# Autodesk Inventor assembly: Chassis Frame Layout
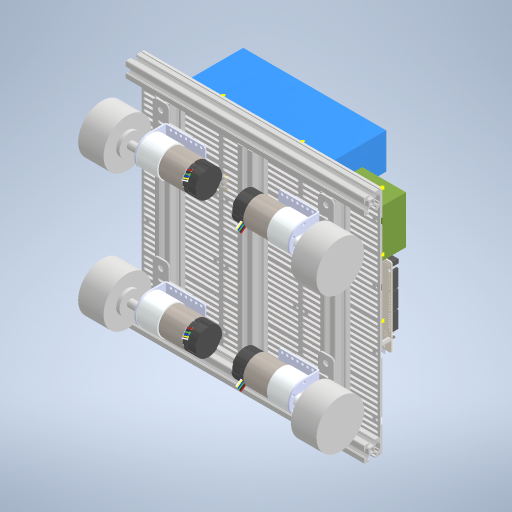
[picture p0: Inventor's stored thumbnail of the model, 512x512]
Saved by Autodesk Inventor 2024 (Build 280153000, 153)
## iProperties
Created: 2023-10-20
Part Number: Chassis Frame Layout
Document SubType Name: Assembly
Designer: olson
Author: olson
## Documents named in this file (20)
- C:\Users\olson\OneDrive\Documents\Senior Year\FALL 2023\ECE 4961 - Capstone 1\Detail Design\Chassis Frame\CAD Models\Chassis Frame Layout.iam
- C:\Users\olson\OneDrive\Documents\Senior Year\FALL 2023\ECE 4961 - Capstone 1\Detail Design\Chassis Frame\CAD Models\Extruded Alumnium 250mm.ipt
- C:\Users\olson\OneDrive\Documents\Senior Year\FALL 2023\ECE 4961 - Capstone 1\Detail Design\Chassis Frame\CAD Models\Extruded Alumnium 300mm.ipt
- C:\Users\olson\OneDrive\Documents\Senior Year\FALL 2023\ECE 4961 - Capstone 1\Detail Design\Chassis Frame\CAD Models\60mm Wheel.ipt
- C:\Users\olson\OneDrive\Documents\Senior Year\FALL 2023\ECE 4961 - Capstone 1\Detail Design\Chassis Frame\CAD Models\60mm Wheel hub.ipt
- C:\Users\olson\OneDrive\Documents\Senior Year\FALL 2023\ECE 4961 - Capstone 1\Detail Design\Chassis Frame\CAD Models\Motor Attachment.ipt
- C:\Users\olson\OneDrive\Documents\Senior Year\FALL 2023\ECE 4961 - Capstone 1\Detail Design\Chassis Frame\CAD Models\pololu-stamped-aluminum-l-bracket-for-37d-mm-metal-gearmotors.ipt
- C:\Users\olson\OneDrive\Documents\Senior Year\FALL 2023\ECE 4961 - Capstone 1\Detail Design\Chassis Frame\CAD Models\37d-gearmotor-10.ipt
- C:\Users\olson\OneDrive\Documents\Senior Year\FALL 2023\ECE 4961 - Capstone 1\Detail Design\Trays\Tray.ipt
- C:\Users\olson\OneDrive\Documents\Senior Year\FALL 2023\ECE 4961 - Capstone 1\Detail Design\Trays\Tray middle.ipt
- C:\Users\olson\OneDrive\Documents\Senior Year\FALL 2023\ECE 4961 - Capstone 1\Detail Design\Trays\connector.ipt
- C:\Users\olson\OneDrive\Documents\Senior Year\FALL 2023\ECE 4961 - Capstone 1\Detail Design\Trays\Mock Battery.ipt
- C:\Users\olson\OneDrive\Documents\Senior Year\FALL 2023\ECE 4961 - Capstone 1\Detail Design\Trays\Mock Charger.ipt
- C:\Users\olson\OneDrive\Documents\Senior Year\FALL 2023\ECE 4961 - Capstone 1\Detail Design\Trays\Mock Gyro-Acc.ipt
- C:\Users\olson\OneDrive\Documents\Senior Year\FALL 2023\ECE 4961 - Capstone 1\Detail Design\Trays\Mock I2C Bus.ipt
- C:\Users\olson\OneDrive\Documents\Senior Year\FALL 2023\ECE 4961 - Capstone 1\Detail Design\Trays\Mock Motor Driver.ipt
- C:\Users\olson\OneDrive\Documents\Senior Year\FALL 2023\ECE 4961 - Capstone 1\Detail Design\Trays\Mock PCB.ipt
- C:\Users\olson\OneDrive\Documents\Senior Year\FALL 2023\ECE 4961 - Capstone 1\Jetson_Nano_2GB_DevKit_P3541_3D_STEP_Model_nv\675_13541_batuu_dev_kit_top_ass_asm\675_13541_batuu_dev_kit_top_ass_asm.iam
- C:\Users\olson\OneDrive\Documents\Senior Year\FALL 2023\ECE 4961 - Capstone 1\Ardunio Mega\ArduinoMega.ipt
- C:\Users\olson\OneDrive\Documents\Senior Year\FALL 2023\ECE 4961 - Capstone 1\Detail Design\Trays\Mock Spacer.ipt
## Components (60 placed, 19 different names)
1. Extruded Alumnium 250mm:2 — Flush:3, Mate:5, Flush:4, Mate:18, Mate:19, Flush:19, Flush:20, Flush:21, Flush:24, Mate:26, Mate:33
2. Extruded Alumnium 250mm:1 — Flush:1, Flush:2, Mate:4, Flush:5, Mate:6, Flush:6, Mate:16, Mate:17, Flush:17, Flush:18, Flush:22, Flush:23, Mate:24, Mate:31
3. Extruded Alumnium 300mm:2 — Flush:5, Mate:6, Flush:6, Flush:7, Mate:7, Flush:8, Mate:74, Flush:33, Flush:34, Mate:75, Flush:35, Mate:77, Flush:36, Flush:37, Flush:48
4. Extruded Alumnium 300mm:1 — Flush:1, Flush:2, Mate:4, Flush:3, Mate:5, Flush:4, Mate:20, Flush:25, Flush:26, Mate:21, Flush:27, Mate:23, Flush:28, Flush:29, Flush:38
5. Extruded Alumnium 250mm:3 — Flush:7, Mate:7, Flush:8, Mate:25, Mate:32
6. 37d-gearmotor-10:5
7. pololu-stamped-aluminum-l-bracket-for-37d-mm-metal-gearmotors:2 — Mate:9, Flush:9, Flush:10
8. Motor Attachment:5 — Mate:9, Flush:9, Flush:10, Mate:16, Flush:18, Flush:23
9. 60mm Wheel:5
10. 60mm Wheel hub:5
11. 37d-gearmotor-10:6
12. pololu-stamped-aluminum-l-bracket-for-37d-mm-metal-gearmotors:3
13. Motor Attachment:6 — Mate:17, Flush:19, Flush:21
14. 60mm Wheel:6
15. 60mm Wheel hub:6
16. 37d-gearmotor-10:7
17. pololu-stamped-aluminum-l-bracket-for-37d-mm-metal-gearmotors:4
18. Motor Attachment:7 — Mate:19, Flush:17, Flush:22
19. 60mm Wheel:7
20. 60mm Wheel hub:7
21. 37d-gearmotor-10:8
22. pololu-stamped-aluminum-l-bracket-for-37d-mm-metal-gearmotors:5
23. Motor Attachment:8 — Mate:18, Flush:20, Flush:24
24. 60mm Wheel:8
25. 60mm Wheel hub:8
26. Tray:1 — Mate:77, Flush:36, Flush:37, Mate:83, Mate:84, Mate:111
27. Tray:2 — Mate:75, Flush:35, Mate:76, Mate:81, Mate:82, Mate:105
28. Tray:3 — Mate:74, Flush:33, Flush:34, Mate:76, Flush:41, Mate:102, Flush:43, Flush:44
29. Tray:4 — Mate:20, Flush:25, Flush:26, Mate:22, Mate:27, Flush:30, Mate:47, Flush:39, Mate:103, Flush:45, Flush:46
30. Tray:5 — Mate:21, Flush:27, Mate:22, Mate:28, Mate:46, Mate:49, Mate:87
31. Tray:6 — Mate:23, Flush:28, Flush:29, Mate:30, Flush:31, Mate:48, Mate:112, Mate:113, Mate:114
32. Tray middle:1 — Mate:31, Mate:34, Flush:32, Mate:37, Mate:85, Mate:86, Mate:109
33. Tray middle:2 — Mate:32, Mate:35, Mate:37, Mate:38, Mate:59, Mate:106
34. Tray middle:3 — Mate:33, Mate:36, Mate:38, Mate:58, Mate:90
35. Tray middle:4 — Mate:24, Mate:27, Flush:30, Mate:29, Mate:34, Flush:32
36. Tray middle:5 — Mate:25, Mate:28, Mate:29, Mate:35, Mate:69, Mate:70
37. Tray middle:6 — Mate:26, Mate:30, Flush:31, Mate:36, Mate:53, Mate:54, Flush:50
38. connector:1 — Mate:48, Mate:49
39. connector:3 — Mate:46, Mate:47
40. connector:4 — Mate:53, Mate:54
41. connector:8 — Mate:58, Mate:59
42. connector:9 — Mate:69, Mate:70
43. connector:12 — Mate:83, Mate:84
44. connector:14 — Mate:81, Mate:82
45. connector:15 — Mate:85, Mate:86
46. Mock Battery:1 — Mate:87, Flush:38, Flush:39, Mate:107, Flush:49
47. Mock Charger:1 — Flush:41, Mate:105, Flush:48, Mate:110, Flush:51
48. Mock Gyro-Acc:1 — Mate:111
49. Mock I2C Bus:1 — Mate:114
50. Mock I2C Bus:2 — Mate:112
51. Mock I2C Bus:3 — Mate:113
52. Mock Motor Driver:1 — Mate:102, Flush:43, Flush:44, Mate:108
53. Mock Motor Driver:2 — Mate:103, Flush:45, Flush:46
54. 675_13541_batuu_dev_kit_top_ass_asm:1 [sub-assembly] — Mate:109, Mate:110, Flush:51
55. ArduinoMega:1 — Mate:90, Mate:92, Mate:93, Mate:94, Mate:95, Mate:96, Mate:97, Flush:50
56. ArduinoMega:2 — Mate:98, Mate:99, Mate:108
57. Mock Spacer:2 — Mate:94, Mate:95, Mate:99
58. Mock Spacer:6 — Mate:92, Mate:93
59. Mock Spacer:8 — Mate:96, Mate:97, Mate:98
60. Mock PCB:1 — Mate:106, Mate:107, Flush:49
## Relationships (138: Mate 78, Flush 48, RevoluteJoint 12)
- [Mate]: Extruded Alumnium 300mm:1
- Flush:1: Extruded Alumnium 250mm:1 ↔ Extruded Alumnium 300mm:1
- Flush:2 (36 mm): Extruded Alumnium 250mm:1 ↔ Extruded Alumnium 300mm:1
- Mate:4: Extruded Alumnium 250mm:1 ↔ Extruded Alumnium 300mm:1
- Flush:3: Extruded Alumnium 250mm:2 ↔ Extruded Alumnium 300mm:1
- Mate:5: Extruded Alumnium 250mm:2 ↔ Extruded Alumnium 300mm:1
- Flush:4 (36 mm): Extruded Alumnium 250mm:2 ↔ Extruded Alumnium 300mm:1
- Flush:5: Extruded Alumnium 250mm:1 ↔ Extruded Alumnium 300mm:2
- Mate:6: Extruded Alumnium 250mm:1 ↔ Extruded Alumnium 300mm:2
- Flush:6 (36 mm): Extruded Alumnium 250mm:1 ↔ Extruded Alumnium 300mm:2
- Flush:7: Extruded Alumnium 300mm:2 ↔ Extruded Alumnium 250mm:3
- Mate:7: Extruded Alumnium 300mm:2 ↔ Extruded Alumnium 250mm:3
- Flush:8 (140 mm): Extruded Alumnium 300mm:2 ↔ Extruded Alumnium 250mm:3
- [Mate]: 37d-gearmotor-10:5 ↔ pololu-stamped-aluminum-l-bracket-for-37d-mm-metal-gearmotors:2
- [RevoluteJoint]: 37d-gearmotor-10:5 ↔ pololu-stamped-aluminum-l-bracket-for-37d-mm-metal-gearmotors:2
- [RevoluteJoint]: 37d-gearmotor-10:5 ↔ 60mm Wheel hub:5
- [RevoluteJoint]: 60mm Wheel:5 ↔ 60mm Wheel hub:5
- Mate:9: pololu-stamped-aluminum-l-bracket-for-37d-mm-metal-gearmotors:2 ↔ Motor Attachment:5
- Flush:9: pololu-stamped-aluminum-l-bracket-for-37d-mm-metal-gearmotors:2 ↔ Motor Attachment:5
- Flush:10 (-16.5 mm): pololu-stamped-aluminum-l-bracket-for-37d-mm-metal-gearmotors:2 ↔ Motor Attachment:5
- [Mate]: 37d-gearmotor-10:6 ↔ pololu-stamped-aluminum-l-bracket-for-37d-mm-metal-gearmotors:3
- [RevoluteJoint]: 37d-gearmotor-10:6 ↔ pololu-stamped-aluminum-l-bracket-for-37d-mm-metal-gearmotors:3
- [RevoluteJoint]: 37d-gearmotor-10:6 ↔ 60mm Wheel hub:6
- [RevoluteJoint]: 60mm Wheel:6 ↔ 60mm Wheel hub:6
- [Mate]: pololu-stamped-aluminum-l-bracket-for-37d-mm-metal-gearmotors:3 ↔ Motor Attachment:6
- [Flush]: pololu-stamped-aluminum-l-bracket-for-37d-mm-metal-gearmotors:3 ↔ Motor Attachment:6
- [Flush] (-16.5 mm): pololu-stamped-aluminum-l-bracket-for-37d-mm-metal-gearmotors:3 ↔ Motor Attachment:6
- [Mate]: 37d-gearmotor-10:7 ↔ pololu-stamped-aluminum-l-bracket-for-37d-mm-metal-gearmotors:4
- [RevoluteJoint]: 37d-gearmotor-10:7 ↔ pololu-stamped-aluminum-l-bracket-for-37d-mm-metal-gearmotors:4
- [RevoluteJoint]: 37d-gearmotor-10:7 ↔ 60mm Wheel hub:7
- [RevoluteJoint]: 60mm Wheel:7 ↔ 60mm Wheel hub:7
- [Mate]: pololu-stamped-aluminum-l-bracket-for-37d-mm-metal-gearmotors:4 ↔ Motor Attachment:7
- [Flush]: pololu-stamped-aluminum-l-bracket-for-37d-mm-metal-gearmotors:4 ↔ Motor Attachment:7
- [Flush] (-16.5 mm): pololu-stamped-aluminum-l-bracket-for-37d-mm-metal-gearmotors:4 ↔ Motor Attachment:7
- [Mate]: 37d-gearmotor-10:8 ↔ pololu-stamped-aluminum-l-bracket-for-37d-mm-metal-gearmotors:5
- [RevoluteJoint]: 37d-gearmotor-10:8 ↔ pololu-stamped-aluminum-l-bracket-for-37d-mm-metal-gearmotors:5
- [RevoluteJoint]: 37d-gearmotor-10:8 ↔ 60mm Wheel hub:8
- [RevoluteJoint]: 60mm Wheel:8 ↔ 60mm Wheel hub:8
- [Mate]: pololu-stamped-aluminum-l-bracket-for-37d-mm-metal-gearmotors:5 ↔ Motor Attachment:8
- [Flush]: pololu-stamped-aluminum-l-bracket-for-37d-mm-metal-gearmotors:5 ↔ Motor Attachment:8
- [Flush] (-16.5 mm): pololu-stamped-aluminum-l-bracket-for-37d-mm-metal-gearmotors:5 ↔ Motor Attachment:8
- Mate:16: Extruded Alumnium 250mm:1 ↔ Motor Attachment:5
- Mate:17: Extruded Alumnium 250mm:1 ↔ Motor Attachment:6
- Mate:18: Extruded Alumnium 250mm:2 ↔ Motor Attachment:8
- Mate:19: Extruded Alumnium 250mm:2 ↔ Motor Attachment:7
- Flush:17: Extruded Alumnium 250mm:1 ↔ Motor Attachment:7
- Flush:18: Extruded Alumnium 250mm:1 ↔ Motor Attachment:5
- Flush:19: Extruded Alumnium 250mm:2 ↔ Motor Attachment:6
- Flush:20: Extruded Alumnium 250mm:2 ↔ Motor Attachment:8
- Flush:21: Extruded Alumnium 250mm:2 ↔ Motor Attachment:6
- Flush:22: Extruded Alumnium 250mm:1 ↔ Motor Attachment:7
- Flush:23: Extruded Alumnium 250mm:1 ↔ Motor Attachment:5
- Flush:24: Extruded Alumnium 250mm:2 ↔ Motor Attachment:8
- Mate:20: Extruded Alumnium 300mm:1 ↔ Tray:4
- Flush:25: Extruded Alumnium 300mm:1 ↔ Tray:4
- Flush:26: Extruded Alumnium 300mm:1 ↔ Tray:4
- Mate:21: Extruded Alumnium 300mm:1 ↔ Tray:5
- Flush:27: Extruded Alumnium 300mm:1 ↔ Tray:5
- Mate:22: Tray:4 ↔ Tray:5
- Mate:23: Extruded Alumnium 300mm:1 ↔ Tray:6
- Flush:28: Extruded Alumnium 300mm:1 ↔ Tray:6
- Flush:29: Extruded Alumnium 300mm:1 ↔ Tray:6
- Mate:24: Extruded Alumnium 250mm:1 ↔ Tray middle:4
- Mate:25: Extruded Alumnium 250mm:3 ↔ Tray middle:5
- Mate:26: Extruded Alumnium 250mm:2 ↔ Tray middle:6
- Mate:27: Tray:4 ↔ Tray middle:4
- Flush:30: Tray:4 ↔ Tray middle:4
- Mate:28: Tray:5 ↔ Tray middle:5
- Mate:29: Tray middle:4 ↔ Tray middle:5
- Mate:30: Tray:6 ↔ Tray middle:6
- Flush:31: Tray:6 ↔ Tray middle:6
- Mate:31: Extruded Alumnium 250mm:1 ↔ Tray middle:1
- Mate:32: Extruded Alumnium 250mm:3 ↔ Tray middle:2
- Mate:33: Extruded Alumnium 250mm:2 ↔ Tray middle:3
- Mate:34: Tray middle:1 ↔ Tray middle:4
- Mate:35: Tray middle:2 ↔ Tray middle:5
- Mate:36: Tray middle:3 ↔ Tray middle:6
- Flush:32: Tray middle:1 ↔ Tray middle:4
- Mate:37: Tray middle:1 ↔ Tray middle:2
- Mate:38: Tray middle:2 ↔ Tray middle:3
- Mate:46: Tray:5 ↔ connector:3
- Mate:47: Tray:4 ↔ connector:3
- Mate:48: Tray:6 ↔ connector:1
- Mate:49: Tray:5 ↔ connector:1
- Mate:53: Tray middle:6 ↔ connector:4
- Mate:54: Tray middle:6 ↔ connector:4
- Mate:58: Tray middle:3 ↔ connector:8
- Mate:59: Tray middle:2 ↔ connector:8
- Mate:69: Tray middle:5 ↔ connector:9
- Mate:70: Tray middle:5 ↔ connector:9
- Mate:74: Extruded Alumnium 300mm:2 ↔ Tray:3
- Flush:33: Extruded Alumnium 300mm:2 ↔ Tray:3
- Flush:34: Extruded Alumnium 300mm:2 ↔ Tray:3
- Mate:75: Extruded Alumnium 300mm:2 ↔ Tray:2
- Flush:35: Extruded Alumnium 300mm:2 ↔ Tray:2
- Mate:76: Tray:2 ↔ Tray:3
- Mate:77: Extruded Alumnium 300mm:2 ↔ Tray:1
- Flush:36: Extruded Alumnium 300mm:2 ↔ Tray:1
- Flush:37: Extruded Alumnium 300mm:2 ↔ Tray:1
- Mate:81: Tray:2 ↔ connector:14
- Mate:82: Tray:2 ↔ connector:14
- Mate:83: Tray:1 ↔ connector:12
- Mate:84: Tray:1 ↔ connector:12
- Mate:85: Tray middle:1 ↔ connector:15
- Mate:86: Tray middle:1 ↔ connector:15
- Mate:87: Tray:5 ↔ Mock Battery:1
- Flush:38: Extruded Alumnium 300mm:1 ↔ Mock Battery:1
- Flush:39 (74.55 mm): Tray:4 ↔ Mock Battery:1
- Flush:41 (60 mm): Tray:3 ↔ Mock Charger:1
- Mate:90: Tray middle:3 ↔ ArduinoMega:1
- Mate:92: ArduinoMega:1 ↔ Mock Spacer:6
- Mate:93: ArduinoMega:1 ↔ Mock Spacer:6
- Mate:94: ArduinoMega:1 ↔ Mock Spacer:2
- Mate:95: ArduinoMega:1 ↔ Mock Spacer:2
- Mate:96: ArduinoMega:1 ↔ Mock Spacer:8
- Mate:97: ArduinoMega:1 ↔ Mock Spacer:8
- Mate:98: ArduinoMega:2 ↔ Mock Spacer:8
- Mate:99: ArduinoMega:2 ↔ Mock Spacer:2
- Mate:102: Tray:3 ↔ Mock Motor Driver:1
- Flush:43: Tray:3 ↔ Mock Motor Driver:1
- Flush:44 (20 mm): Tray:3 ↔ Mock Motor Driver:1
- Mate:103: Tray:4 ↔ Mock Motor Driver:2
- Flush:45 (20 mm): Tray:4 ↔ Mock Motor Driver:2
- Flush:46: Tray:4 ↔ Mock Motor Driver:2
- Mate:105: Tray:2 ↔ Mock Charger:1
- Flush:48: Extruded Alumnium 300mm:2 ↔ Mock Charger:1
- Mate:106: Tray middle:2 ↔ Mock PCB:1
- Mate:107: Mock Battery:1 ↔ Mock PCB:1
- Flush:49: Mock Battery:1 ↔ Mock PCB:1
- Mate:108 (15 mm): Mock Motor Driver:1 ↔ ArduinoMega:2
- Flush:50 (10 mm): Tray middle:6 ↔ ArduinoMega:1
- Mate:109: Tray middle:1 ↔ 675_13541_batuu_dev_kit_top_ass_asm:1
- Mate:110 (10 mm): Mock Charger:1 ↔ 675_13541_batuu_dev_kit_top_ass_asm:1
- Flush:51 (130 mm): Mock Charger:1 ↔ 675_13541_batuu_dev_kit_top_ass_asm:1
- Mate:111: Tray:1 ↔ Mock Gyro-Acc:1
- Mate:112: Tray:6 ↔ Mock I2C Bus:2
- Mate:113: Tray:6 ↔ Mock I2C Bus:3
- Mate:114: Tray:6 ↔ Mock I2C Bus:1
## Named parameters: d34_d21 = 0 mm, d35_d22 = 0 mm, d36_d23 = 180 deg, d47_d34_d21 = 0 mm, d48_d35_d22 = 0 mm, d49_d36_d23 = 180 deg, d50_d36 = 0 mm, d51_d37 = -90 deg, d52_d38 = 0 mm, d53_d39 = 0 deg, d54_d44 = 0 mm, d55_d45 = 0 mm, d56_d46 = -16.5 mm, d57_d34_d21 = 0 mm, d58_d35_d22 = 0 mm, d59_d36_d23 = 180 deg, d60_d36 = 0 mm, d61_d37 = -90 deg, d62_d38 = 0 mm, d63_d39 = 0 deg, d64_d44 = 0 mm, d65_d45 = 0 mm, d66_d46 = -16.5 mm, d67_d34_d21 = 0 mm, d68_d35_d22 = 0 mm, d69_d36_d23 = 180 deg, d70_d36 = 0 mm, d71_d37 = 90 deg, d72_d38 = 0 mm, d73_d39 = 0 deg, d74_d44 = 0 mm, d75_d45 = 0 mm, d76_d46 = -16.5 mm
